# Autodesk Inventor assembly: wafel_rev2
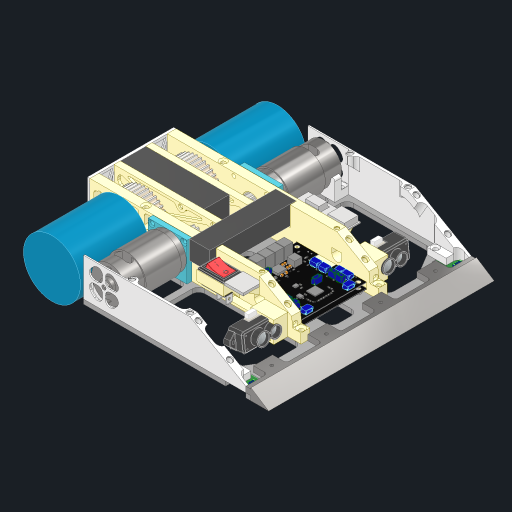
[picture p0: Inventor's stored thumbnail of the model, 512x512]
Saved by Autodesk Inventor 2023 (Build 270158000, 158)
## iProperties
Created: 2024-04-29
Part Number: wafel_rev2
Document SubType Name: Assembly
Designer: szymo
Mass: 970.153 g
Surface Area: 2764.06 cm^2
Volume: 500.252 cm^3
Density: 1.93933 g/cm^3
Author: szymo
## Documents named in this file (27)
- D:\roboilo\robots\codename wafel - australia\3d_parts\rev2_v2\wafel_rev2_v2.iam
- D:\roboilo\robots\codename wafel - australia\3d_parts\rev2_v2\plog.ipt
- D:\roboilo\robots\codename wafel - australia\3d_parts\rev2_v2\smolgear_shaft.ipt
- D:\roboilo\robots\codename wafel - australia\3d_parts\rev2_v2\smolLipo.ipt
- D:\roboilo\robots\codename wafel - australia\3d_parts\rev2_v2\stack.iam
- D:\roboilo\robots\codename wafel - australia\3d_parts\rev2_v2\Switch.ipt
- D:\roboilo\robots\codename wafel - australia\3d_parts\rev2_v2\TFMiniS.ipt
- D:\roboilo\robots\codename wafel - australia\3d_parts\rev2_v2\wheel_axle.iam
- D:\roboilo\robots\codename wafel - australia\3d_parts\rev2_v2\KTIR-Board.ipt
- D:\roboilo\robots\codename wafel - australia\3d_parts\rev2_v2\lipo3s650.ipt
- D:\roboilo\robots\codename wafel - australia\3d_parts\rev2_v2\Design Accelerator\smolGear.iam
- D:\roboilo\robots\codename wafel - australia\3d_parts\rev2_v2\motor_w_gear.iam
- D:\roboilo\robots\codename wafel - australia\3d_parts\rev2_v2\base.ipt
- D:\roboilo\robots\codename wafel - australia\3d_parts\rev2_v2\wheel.ipt
- D:\roboilo\robots\codename wafel - australia\3d_parts\rev2_v2\left_hold.ipt
- D:\roboilo\robots\codename wafel - australia\3d_parts\rev2_v2\front_motur_holder.ipt
- D:\roboilo\robots\codename wafel - australia\3d_parts\rev2_v2\front_motur_holder_MIR.ipt
- D:\roboilo\robots\codename wafel - australia\3d_parts\rev2_v2\right_gear_holder.ipt
- D:\roboilo\robots\codename wafel - australia\3d_parts\rev2_v2\right_gear_holder_MIR.ipt
- D:\roboilo\robots\codename wafel - australia\3d_parts\rev2_v2\interface_board.ipt
- D:\roboilo\robots\codename wafel - australia\3d_parts\rev2_v2\back.ipt
- D:\roboilo\robots\codename wafel - australia\3d_parts\rev2_v2\oled.ipt
- D:\roboilo\robots\codename wafel - australia\3d_parts\rev2_v2\right_side.ipt
- D:\roboilo\robots\codename wafel - australia\3d_parts\rev2_v2\right_side_MIR.ipt
- D:\roboilo\robots\codename wafel - australia\3d_parts\rev2_v2\frobt.ipt
- D:\roboilo\robots\codename wafel - australia\3d_parts\rev2_v2\ceil.ipt
- D:\roboilo\robots\codename wafel - australia\3d_parts\rev2_v2\left_hold_MIR.ipt
## Components (33 placed, 26 different names)
1. base:1 — Flush:1, Mate:2, Tangent:1, Angle:1, Tangent:2, Mate:5, Angle:2, Tangent:6, Flush:7, Flush:8, Tangent:7, Mate:7, Flush:9, Flush:17, Flush:21, Flush:22, Mate:14, Mate:25, Mate:26, Mate:27, Mate:28, Flush:37, Flush:38, Flush:39, Flush:40, Tangent:8, Angle:5, Tangent:10
2. plog:1 — Flush:1, Mate:2, Mate:9, Angle:3, Angle:4
3. left_hold:1 — Mate:17, Mate:19, Flush:23, Flush:35, Flush:36, Mate:32
4. left_hold_MIR:1 — Flush:47, Mate:30, Mate:31
5. right_gear_holder_MIR:1
6. right_gear_holder:1 — Flush:17
7. front_motur_holder_MIR:1 — Mate:20, Mate:33
8. front_motur_holder:1 — Flush:49
9. TFMiniS:1 — Mate:14, Angle:3, Angle:4, Symmetry:15, Symmetry:16, Symmetry:17
10. wheel_axle:1 [sub-assembly] — Flush:2, Flush:3, Mate:3, Mate:4, Tangent:1, Tangent:5, Symmetry:3, Symmetry:4, Mate:6
11. smolGear:1 [sub-assembly] — Flush:3, Tangent:4, Tangent:5, Symmetry:5, Symmetry:12, Mate:12
12. wheel:1 — Mate:3, Mate:4, Angle:1, Tangent:6, Symmetry:1, Symmetry:2
13. motor_w_gear:1 [sub-assembly] — Flush:2, Tangent:2, Tangent:4, Angle:2, Tangent:7, Flush:49
14. motor_w_gear:2 [sub-assembly] — Flush:50, Flush:51, Tangent:8, Tangent:9, Angle:5, Tangent:10, Mate:33
15. wheel_axle:2 [sub-assembly] — Symmetry:3, Symmetry:4, Flush:51
16. TFMiniS:2 — Symmetry:15, Symmetry:16, Symmetry:17
17. smolGear:2 [sub-assembly] — Symmetry:5, Symmetry:12, Flush:50, Tangent:9
18. wheel:2 — Symmetry:1, Symmetry:2
19. lipo3s650:1 — Mate:5, Flush:7, Flush:8, Mate:6
20. smolLipo:1 — Mate:17, Mate:32
21. smolgear_shaft:1 — Symmetry:13, Symmetry:14
22. smolgear_shaft:2 — Mate:12, Symmetry:13, Symmetry:14
23. stack:1 [sub-assembly] — Mate:7, Flush:9, Mate:9
24. Switch:1 — Flush:46, Mate:29, Flush:48, Mate:30
25. KTIR-Board:1 — Mate:27, Mate:28, Flush:38
26. KTIR-Board:2 — Mate:25, Mate:26, Flush:39
27. interface_board:1 — Mate:19, Flush:23, Mate:20, Flush:35, Flush:36
28. back:1 — Flush:21, Flush:22
29. oled:1 — Flush:46, Mate:29, Flush:47, Flush:48, Mate:31
30. right_side:1 — Flush:37, Flush:40, Flush:41, Flush:45
31. right_side_MIR:1
32. frobt:1 — Flush:41
33. ceil:1 — Flush:45
## Relationships (70: Flush 24, Mate 21, Symmetry 11, Tangent 9, Angle 5)
- Flush:1: base:1 ↔ plog:1
- Mate:2: base:1 ↔ plog:1
- Flush:2: wheel_axle:1 ↔ motor_w_gear:1
- Flush:3: wheel_axle:1 ↔ smolGear:1
- Mate:3: wheel_axle:1 ↔ wheel:1
- Mate:4 (2 mm): wheel_axle:1 ↔ wheel:1
- Tangent:1 (3 mm): base:1 ↔ wheel_axle:1
- Angle:1 (0 deg): base:1 ↔ wheel:1
- Tangent:2 (1 mm): base:1 ↔ motor_w_gear:1
- Tangent:4: smolGear:1 ↔ motor_w_gear:1
- Tangent:5: wheel_axle:1 ↔ smolGear:1
- Mate:5: base:1 ↔ lipo3s650:1
- Angle:2 (0 deg): base:1 ↔ motor_w_gear:1
- Tangent:6 (2.5 mm): base:1 ↔ wheel:1
- Symmetry:1: wheel:1 ↔ wheel:2
- Symmetry:2: wheel:1 ↔ wheel:2
- Symmetry:3: wheel_axle:1 ↔ wheel_axle:2
- Symmetry:4: wheel_axle:1 ↔ wheel_axle:2
- Symmetry:5: smolGear:1 ↔ smolGear:2
- Symmetry:12: smolGear:1 ↔ smolGear:2
- Flush:7 (79 mm): base:1 ↔ lipo3s650:1
- Flush:8: base:1 ↔ lipo3s650:1
- Tangent:7 (1 mm): base:1 ↔ motor_w_gear:1
- Mate:6 (1 mm): wheel_axle:1 ↔ lipo3s650:1
- Mate:7 (2 mm): base:1 ↔ stack:1
- Flush:9 (61.5 mm): base:1 ↔ stack:1
- Mate:9 (10 mm): plog:1 ↔ stack:1
- Flush:17: base:1 ↔ right_gear_holder:1
- Mate:12: smolGear:1 ↔ smolgear_shaft:2
- Symmetry:13: smolgear_shaft:1 ↔ smolgear_shaft:2
- Symmetry:14: smolgear_shaft:1 ↔ smolgear_shaft:2
- Flush:21: base:1 ↔ back:1
- Flush:22: base:1 ↔ back:1
- Mate:14: base:1 ↔ TFMiniS:1
- Angle:3 (353.5 deg): plog:1 ↔ TFMiniS:1
- Angle:4 (0 deg): plog:1 ↔ TFMiniS:1
- Symmetry:15: TFMiniS:1 ↔ TFMiniS:2
- Symmetry:16: TFMiniS:1 ↔ TFMiniS:2
- Symmetry:17: TFMiniS:1 ↔ TFMiniS:2
- Mate:17: left_hold:1 ↔ smolLipo:1
- Mate:19: left_hold:1 ↔ interface_board:1
- Flush:23 (-5 mm): left_hold:1 ↔ interface_board:1
- Mate:20 (5 mm): front_motur_holder_MIR:1 ↔ interface_board:1
- Flush:35: left_hold:1 ↔ interface_board:1
- Flush:36: left_hold:1 ↔ interface_board:1
- Mate:25 (0.5 mm): base:1 ↔ KTIR-Board:2
- Mate:26 (0.5 mm): base:1 ↔ KTIR-Board:2
- Mate:27 (0.5 mm): base:1 ↔ KTIR-Board:1
- Mate:28 (0.5 mm): base:1 ↔ KTIR-Board:1
- Flush:37: base:1 ↔ right_side:1
- Flush:38: base:1 ↔ KTIR-Board:1
- Flush:39: base:1 ↔ KTIR-Board:2
- Flush:40: base:1 ↔ right_side:1
- Flush:41: right_side:1 ↔ frobt:1
- Flush:45: right_side:1 ↔ ceil:1
- Flush:46: Switch:1 ↔ oled:1
- Mate:29 (0.5 mm): Switch:1 ↔ oled:1
- Flush:47 (-5 mm): left_hold_MIR:1 ↔ oled:1
- Flush:48: Switch:1 ↔ oled:1
- Mate:30 (-2 mm): left_hold_MIR:1 ↔ Switch:1
- Mate:31: left_hold_MIR:1 ↔ oled:1
- Flush:49: front_motur_holder:1 ↔ motor_w_gear:1
- Mate:32: left_hold:1 ↔ smolLipo:1
- Flush:50: motor_w_gear:2 ↔ smolGear:2
- Flush:51: motor_w_gear:2 ↔ wheel_axle:2
- Tangent:8 (1 mm): base:1 ↔ motor_w_gear:2
- Tangent:9: motor_w_gear:2 ↔ smolGear:2
- Angle:5 (0 deg): base:1 ↔ motor_w_gear:2
- Tangent:10 (1 mm): base:1 ↔ motor_w_gear:2
- Mate:33: front_motur_holder_MIR:1 ↔ motor_w_gear:2
